# Autodesk Inventor assembly: Automoblox Assembly
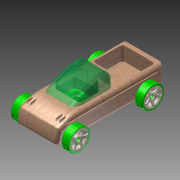
[picture p0: Inventor's stored thumbnail of the model, 180x180]
Saved by Autodesk Inventor 2015 (Build 190159000, 159)
## iProperties
Created: 2018-02-22
Part Number: Automoblox Assembly
Document SubType Name: Assembly
Designer: Administrator
Author: Administrator
## Documents named in this file (12)
- L:\IED 9th\Automoblox\7.4 Exact Parts\Automoblox Assembly.iam
- L:\IED 9th\Automoblox\7.4 Exact Parts\T9 Passenger Section.ipt
- L:\IED 9th\Automoblox\7.4 Exact Parts\T9 One Block Socket.ipt
- L:\IED 9th\Automoblox\7.4 Exact Parts\T9 Two Block Socket.ipt
- L:\IED 9th\Automoblox\7.4 Exact Parts\T9 Passenger Base.ipt
- L:\IED 9th\Automoblox\7.4 Exact Parts\T9 Connector.ipt
- L:\IED 9th\Automoblox\7.4 Exact Parts\T9 Windshield.ipt
- L:\IED 9th\Automoblox\7.4 Exact Parts\T9 Bed.ipt
- L:\IED 9th\Automoblox\7.4 Exact Parts\T9 Axle.ipt
- L:\IED 9th\Automoblox\7.4 Exact Parts\T9 Front.ipt
- L:\IED 9th\Automoblox\7.4 Exact Parts\T9 Wheel.ipt
- L:\IED 9th\Automoblox\7.4 Exact Parts\T9 Tire.ipt
## Components (23 placed, 11 different names)
1. T9 Passenger Section:1 — Mate:7, Mate:8, Mate:9, Mate:10, Mate:11, Mate:12, Mate:13, Mate:14, Mate:15, Mate:16, Mate:17, Mate:18, Flush:2, Mate:30, Flush:3, Flush:4, Mate:31, Flush:5
2. T9 One Block Socket:1 — Mate:12, Mate:13, Mate:14, Mate:25, Flush:1, Mate:26
3. T9 One Block Socket:2 — Mate:19, Mate:20, Mate:21, Mate:27, Mate:28, Mate:29
4. T9 Two Block Socket:1 — Mate:7, Mate:8, Mate:15
5. T9 Two Block Socket:2 — Mate:22, Mate:23, Mate:24
6. T9 Passenger Base:1 — Mate:9, Mate:10, Mate:11
7. T9 Connector:1 — Mate:25, Flush:1, Mate:26
8. T9 Connector:2 — Mate:27, Mate:28, Mate:29
9. T9 Windshield:1 — Mate:16, Mate:17, Mate:18
10. T9 Bed:1 — Mate:19, Mate:20, Mate:21, Insert:1, Insert:2, Flush:4, Mate:31, Flush:5
11. T9 Axle:1 — Insert:4, Insert:8
12. T9 Axle:2 — Insert:2, Insert:7
13. T9 Axle:3 — Insert:3, Insert:5
14. T9 Axle:4 — Insert:1, Insert:6
15. T9 Front:1 — Insert:3, Insert:4, Mate:22, Mate:23, Mate:24, Flush:2, Mate:30, Flush:3
16. T9 Wheel:1 — Insert:8, Mate:32, Flush:6
17. T9 Wheel:2 — Insert:7, Flush:7, Mate:33
18. T9 Wheel:3 — Insert:6, Flush:9, Mate:35
19. T9 Wheel:4 — Insert:5, Mate:34, Flush:8
20. T9 Tire:1 — Mate:32, Flush:6
21. T9 Tire:2 — Flush:7, Mate:33
22. T9 Tire:3 — Mate:34, Flush:8
23. T9 Tire:4 — Flush:9, Mate:35
## Relationships (46: Mate 29, Flush 9, Insert 8)
- Mate:7: T9 Passenger Section:1 ↔ T9 Two Block Socket:1
- Mate:8: T9 Passenger Section:1 ↔ T9 Two Block Socket:1
- Mate:9: T9 Passenger Section:1 ↔ T9 Passenger Base:1
- Mate:10: T9 Passenger Section:1 ↔ T9 Passenger Base:1
- Mate:11: T9 Passenger Section:1 ↔ T9 Passenger Base:1
- Mate:12: T9 Passenger Section:1 ↔ T9 One Block Socket:1
- Mate:13: T9 Passenger Section:1 ↔ T9 One Block Socket:1
- Mate:14: T9 Passenger Section:1 ↔ T9 One Block Socket:1
- Mate:15: T9 Passenger Section:1 ↔ T9 Two Block Socket:1
- Mate:16: T9 Passenger Section:1 ↔ T9 Windshield:1
- Mate:17: T9 Passenger Section:1 ↔ T9 Windshield:1
- Mate:18: T9 Passenger Section:1 ↔ T9 Windshield:1
- Mate:19: T9 One Block Socket:2 ↔ T9 Bed:1
- Mate:20: T9 One Block Socket:2 ↔ T9 Bed:1
- Mate:21: T9 One Block Socket:2 ↔ T9 Bed:1
- Insert:1: T9 Bed:1 ↔ T9 Axle:4
- Insert:2: T9 Bed:1 ↔ T9 Axle:2
- Insert:3: T9 Axle:3 ↔ T9 Front:1
- Insert:4: T9 Axle:1 ↔ T9 Front:1
- Mate:22: T9 Two Block Socket:2 ↔ T9 Front:1
- Mate:23: T9 Two Block Socket:2 ↔ T9 Front:1
- Mate:24: T9 Two Block Socket:2 ↔ T9 Front:1
- Mate:25: T9 One Block Socket:1 ↔ T9 Connector:1
- Flush:1: T9 One Block Socket:1 ↔ T9 Connector:1
- Mate:26: T9 One Block Socket:1 ↔ T9 Connector:1
- Mate:27: T9 One Block Socket:2 ↔ T9 Connector:2
- Mate:28: T9 One Block Socket:2 ↔ T9 Connector:2
- Mate:29: T9 One Block Socket:2 ↔ T9 Connector:2
- Flush:2: T9 Passenger Section:1 ↔ T9 Front:1
- Mate:30: T9 Passenger Section:1 ↔ T9 Front:1
- Flush:3: T9 Passenger Section:1 ↔ T9 Front:1
- Flush:4: T9 Passenger Section:1 ↔ T9 Bed:1
- Mate:31: T9 Passenger Section:1 ↔ T9 Bed:1
- Flush:5: T9 Passenger Section:1 ↔ T9 Bed:1
- Insert:5: T9 Axle:3 ↔ T9 Wheel:4
- Insert:6: T9 Axle:4 ↔ T9 Wheel:3
- Insert:7: T9 Axle:2 ↔ T9 Wheel:2
- Insert:8: T9 Axle:1 ↔ T9 Wheel:1
- Mate:32: T9 Wheel:1 ↔ T9 Tire:1
- Flush:6: T9 Wheel:1 ↔ T9 Tire:1
- Flush:7: T9 Wheel:2 ↔ T9 Tire:2
- Mate:33: T9 Wheel:2 ↔ T9 Tire:2
- Mate:34: T9 Wheel:4 ↔ T9 Tire:3
- Flush:8: T9 Wheel:4 ↔ T9 Tire:3
- Flush:9: T9 Wheel:3 ↔ T9 Tire:4
- Mate:35: T9 Wheel:3 ↔ T9 Tire:4
